# Autodesk Inventor assembly: Catapult Launcher
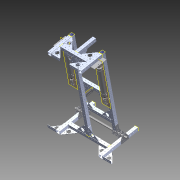
[picture p0: Inventor's stored thumbnail of the model, 180x180]
Saved by Autodesk Inventor 2014 (Build 180170000, 170)
## iProperties
Created: 2014-01-17
Part Number: Catapult Launcher
Document SubType Name: Assembly
Designer: Andrew Toennies
Mass: 1552.27 g
Surface Area: 5150.08 cm^2
Volume: 383.1 cm^3
Density: 4.05187 g/cm^3
Author: Andrew Toennies
## Documents named in this file (18)
- C:\Users\Andrew Toennies\Documents\GitHub\2014buildCAD\New Shooter\Catapult Launcher.iam
- C:\Users\Andrew Toennies\Documents\GitHub\2014buildCAD\New Shooter\Vex Pro 1x1 rectangular tubing 7 in length.ipt
- C:\Users\Andrew Toennies\Documents\GitHub\2014buildCAD\New Shooter\Vex Pro Side Bearing Gusset - OUT OF STOCK 1192014.ipt
- C:\Users\Andrew Toennies\Documents\GitHub\2014buildCAD\New Shooter\Vex Pro Corner Gusset - IN STOCK 1192014.ipt
- C:\Users\Andrew Toennies\Documents\GitHub\2014buildCAD\New Shooter\Bearing ID 0.500 Hex OD 1.125.ipt
- C:\Users\Andrew Toennies\Documents\GitHub\2014buildCAD\New Shooter\Shaft (Steel 0.500 Hex).ipt
- C:\Users\Andrew Toennies\Documents\GitHub\2014buildCAD\New Shooter\Vex Pro 1x1 rectangular tubing 27 in length.ipt
- C:\Users\Andrew Toennies\Documents\GitHub\2014buildCAD\New Shooter\Vex Pro 1x1 rectangular tubing 3 in length.ipt
- C:\Users\Andrew Toennies\Documents\GitHub\2014buildCAD\New Shooter\Vex Pro 1x1 rectangular tubing 11 in length.ipt
- C:\Users\Andrew Toennies\Documents\GitHub\2014buildCAD\New Shooter\1.5 in bore 6 in stroke cylinder - BIMBA\176-DP(D-229)(F,D-231-1).iam
- C:\Users\Andrew Toennies\Documents\GitHub\2014buildCAD\New Shooter\Aluminum Plate (0.125).ipt
- C:\Users\Andrew Toennies\Documents\GitHub\2014buildCAD\New Shooter\1.5 in bore 6 in stroke cylinder - BIMBA\D-14826.ipt
- C:\Users\Andrew Toennies\Documents\GitHub\2014buildCAD\New Shooter\1.5 in bore 6 in stroke cylinder - BIMBA\D-9969.ipt
- C:\Users\Andrew Toennies\Documents\GitHub\2014buildCAD\New Shooter\Vex Pro End Bearing Mount - IN STOCK 1192014.ipt
- C:\Users\Andrew Toennies\Documents\GitHub\2014buildCAD\New Shooter\Vex Pro 1x1 rectangular tubing 13 in length.ipt
- C:\Users\Andrew Toennies\Documents\GitHub\2014buildCAD\New Shooter\Vex Pro 1x1 rectangular tubing 25 in length.ipt
- C:\Users\Andrew Toennies\Documents\GitHub\2014buildCAD\New Shooter\0.5625 in bore 2 in stroke compact cylinder - BIMBA\FO-022.iam
- C:\Users\Andrew Toennies\Documents\GitHub\2014buildCAD\New Shooter\Vex Pro 1x1 rectangular tubing 8 in length.ipt
## Components (53 placed, 17 different names)
1. Shaft (Steel 0.500 Hex):1 — Mate:34, Mate:35, Flush:25, Mate:227, Mate:228
2. Vex Pro 1x1 rectangular tubing 11 in length:3 — Mate:272, Flush:48, Mate:274, Flush:49, Mate:277, Flush:50, Mate:290, Mate:291, Mate:293, Flush:57, Mate:298, Flush:60
3. Vex Pro Corner Gusset - IN STOCK 1192014:15 — Mate:273, Mate:274, Flush:49, Mate:275
4. Vex Pro Corner Gusset - IN STOCK 1192014:16 — Mate:276, Mate:277, Flush:50
5. Vex Pro 1x1 rectangular tubing 13 in length:1 — Mate:278, Flush:51, Mate:280, Flush:52, Mate:281, Mate:284, Flush:55, Mate:294, Mate:296
6. Vex Pro 1x1 rectangular tubing 25 in length:1 — Mate:284, Flush:55, Mate:285, Mate:287, Mate:288, Mate:289, Flush:56, Mate:292, Mate:295, Flush:58, Mate:297, Flush:59, Flush:61, Mate:300
7. FO-022:1 [sub-assembly] — Mate:285, Mate:287, Mate:288
8. Vex Pro Corner Gusset - IN STOCK 1192014:17 — Mate:289, Mate:290, Flush:56, Mate:291
9. Vex Pro Corner Gusset - IN STOCK 1192014:18 — Mate:292, Mate:293, Flush:57
10. Vex Pro Corner Gusset - IN STOCK 1192014:19 — Mate:294, Mate:295, Flush:58
11. Vex Pro Corner Gusset - IN STOCK 1192014:20 — Mate:296, Mate:297, Flush:59
12. Vex Pro 1x1 rectangular tubing 8 in length:1 — Mate:298, Flush:60, Flush:61, Mate:299, Flush:62
13. Vex Pro Corner Gusset - IN STOCK 1192014:21 — Mate:299, Mate:300, Flush:62
14. Vex Pro 1x1 rectangular tubing 7 in length:1 — Flush:1, Flush:2, Mate:8, Mate:11, Mate:23, Mate:24, Mate:25, Mate:195, Flush:32, Flush:33, Flush:34, Flush:35, Mate:278, Flush:51, Mate:279
15. Vex Pro 1x1 rectangular tubing 7 in length:2 — Flush:1, Flush:2, Mate:3, Mate:5, Mate:14, Mate:15, Mate:16, Mate:123, Mate:188, Mate:195, Flush:25, Flush:28, Flush:29, Flush:30, Flush:31, Mate:282, Flush:54, Mate:283
16. Vex Pro Side Bearing Gusset - OUT OF STOCK 1192014:1 — Mate:3, Mate:26, Mate:27, Flush:28, Flush:29
17. Vex Pro Side Bearing Gusset - OUT OF STOCK 1192014:2 — Mate:5, Mate:28, Mate:29, Flush:30, Flush:31
18. Vex Pro Side Bearing Gusset - OUT OF STOCK 1192014:3 — Mate:11, Mate:32, Mate:33, Flush:32, Flush:33
19. Vex Pro Side Bearing Gusset - OUT OF STOCK 1192014:4 — Mate:8, Mate:30, Mate:31, Flush:34, Flush:35
20. Vex Pro Corner Gusset - IN STOCK 1192014:1 — Mate:281, Mate:282, Flush:54, Mate:283
21. Vex Pro Corner Gusset - IN STOCK 1192014:2 — Mate:14, Mate:15, Mate:16, Flush:53
22. Vex Pro Corner Gusset - IN STOCK 1192014:3 — Mate:279, Mate:280, Flush:52
23. Vex Pro Corner Gusset - IN STOCK 1192014:4 — Mate:23, Mate:24, Mate:25
24. Bearing ID 0.500 Hex OD 1.125:1 — Mate:28, Mate:29, Flush:3, Flush:5
25. Bearing ID 0.500 Hex OD 1.125:2 — Mate:26, Mate:27, Flush:3, Mate:34, Mate:35
26. Bearing ID 0.500 Hex OD 1.125:3 — Mate:30, Mate:31, Flush:4
27. Bearing ID 0.500 Hex OD 1.125:4 — Mate:32, Mate:33, Flush:4, Flush:5, Mate:69
28. Vex Pro Corner Gusset - IN STOCK 1192014:14 — Mate:250, Mate:251, Flush:45, Mate:271
29. Vex Pro Corner Gusset - IN STOCK 1192014:13 — Mate:252, Mate:253, Flush:46
30. Vex Pro Corner Gusset - IN STOCK 1192014:12 — Mate:248, Mate:249, Flush:44
31. Vex Pro Corner Gusset - IN STOCK 1192014:11 — Mate:243, Flush:43, Mate:244
32. Vex Pro 1x1 rectangular tubing 11 in length:1 — Mate:191, Flush:42, Mate:250, Mate:253, Flush:46, Mate:267
33. Vex Pro 1x1 rectangular tubing 11 in length:2 — Flush:41, Mate:242, Mate:243, Flush:43, Mate:246, Mate:248, Flush:44
34. D-9969:1 — Mate:164, Mate:165, Mate:166, Mate:198, Flush:36, Mate:270
35. D-14826:1 — Mate:164, Mate:169, Mate:170, Flush:37, Mate:247, Mate:265, Mate:266
36. Vex Pro End Bearing Mount - IN STOCK 1192014:4 — Mate:229, Mate:230, Mate:231, Mate:232, Mate:246
37. Vex Pro End Bearing Mount - IN STOCK 1192014:3 — Mate:217, Mate:218, Mate:219, Mate:220, Mate:221
38. Vex Pro End Bearing Mount - IN STOCK 1192014:2 — Mate:233, Mate:234, Mate:235, Mate:236, Mate:245
39. Vex Pro End Bearing Mount - IN STOCK 1192014:1 — Mate:222, Mate:223, Mate:224, Mate:225, Mate:226
40. Vex Pro 1x1 rectangular tubing 27 in length:3 — Mate:198, Mate:229, Mate:230, Mate:231, Mate:233, Mate:234, Mate:235, Flush:27, Flush:36, Flush:41, Mate:242, Mate:244, Mate:251, Flush:45, Mate:267, Mate:270, Mate:271
41. Vex Pro 1x1 rectangular tubing 27 in length:2 — Mate:188, Mate:191, Mate:212, Mate:219, Mate:220, Mate:221, Mate:224, Mate:225, Mate:226, Flush:26, Flush:37, Flush:42, Mate:247, Mate:249, Mate:252
42. Bearing ID 0.500 Hex OD 1.125:5 — Mate:80, Mate:222, Mate:223, Mate:228
43. Bearing ID 0.500 Hex OD 1.125:6 — Mate:80, Mate:217, Mate:218, Mate:227
44. Bearing ID 0.500 Hex OD 1.125:7 — Mate:68, Mate:69, Mate:236, Mate:245
45. Bearing ID 0.500 Hex OD 1.125:8 — Mate:68, Mate:232
46. 176-DP(D-229)(F,D-231-1):1 [sub-assembly] — Mate:153, Mate:154, Mate:155, Mate:165, Mate:166, Mate:171
47. 176-DP(D-229)(F,D-231-1):2 [sub-assembly] — Mate:156, Mate:167, Mate:168, Mate:169, Mate:170, Mate:171, Mate:265, Mate:266
48. Aluminum Plate (0.125):1 — Mate:153, Mate:154, Mate:155, Mate:159, Flush:24
49. Aluminum Plate (0.125):2 — Mate:156, Mate:160, Mate:167, Mate:168, Flush:24, Flush:47
50. Vex Pro 1x1 rectangular tubing 3 in length:2 — Mate:121, Flush:14, Mate:122, Flush:19, Mate:159, Flush:27, Mate:276
51. Vex Pro 1x1 rectangular tubing 3 in length:1 — Flush:13, Mate:118, Mate:119, Mate:120, Mate:123, Flush:19, Mate:160, Mate:212, Flush:26, Flush:47, Mate:272, Flush:48, Mate:273, Mate:275
52. Vex Pro Corner Gusset - IN STOCK 1192014:8 — Flush:13, Mate:118, Mate:119, Mate:120, Flush:17, Flush:53
53. Vex Pro Corner Gusset - IN STOCK 1192014:6 — Mate:121, Flush:14, Mate:122, Flush:17
## Relationships (158: Mate 113, Flush 45)
- Flush:1: Vex Pro 1x1 rectangular tubing 7 in length:1 ↔ Vex Pro 1x1 rectangular tubing 7 in length:2
- Flush:2: Vex Pro 1x1 rectangular tubing 7 in length:1 ↔ Vex Pro 1x1 rectangular tubing 7 in length:2
- Mate:3: Vex Pro 1x1 rectangular tubing 7 in length:2 ↔ Vex Pro Side Bearing Gusset - OUT OF STOCK 1192014:1
- Mate:5: Vex Pro 1x1 rectangular tubing 7 in length:2 ↔ Vex Pro Side Bearing Gusset - OUT OF STOCK 1192014:2
- Mate:8: Vex Pro 1x1 rectangular tubing 7 in length:1 ↔ Vex Pro Side Bearing Gusset - OUT OF STOCK 1192014:4
- Mate:11: Vex Pro 1x1 rectangular tubing 7 in length:1 ↔ Vex Pro Side Bearing Gusset - OUT OF STOCK 1192014:3
- Mate:14: Vex Pro 1x1 rectangular tubing 7 in length:2 ↔ Vex Pro Corner Gusset - IN STOCK 1192014:2
- Mate:15: Vex Pro 1x1 rectangular tubing 7 in length:2 ↔ Vex Pro Corner Gusset - IN STOCK 1192014:2
- Mate:16: Vex Pro 1x1 rectangular tubing 7 in length:2 ↔ Vex Pro Corner Gusset - IN STOCK 1192014:2
- Mate:23: Vex Pro 1x1 rectangular tubing 7 in length:1 ↔ Vex Pro Corner Gusset - IN STOCK 1192014:4
- Mate:24: Vex Pro 1x1 rectangular tubing 7 in length:1 ↔ Vex Pro Corner Gusset - IN STOCK 1192014:4
- Mate:25: Vex Pro 1x1 rectangular tubing 7 in length:1 ↔ Vex Pro Corner Gusset - IN STOCK 1192014:4
- Mate:26: Vex Pro Side Bearing Gusset - OUT OF STOCK 1192014:1 ↔ Bearing ID 0.500 Hex OD 1.125:2
- Mate:27: Vex Pro Side Bearing Gusset - OUT OF STOCK 1192014:1 ↔ Bearing ID 0.500 Hex OD 1.125:2
- Mate:28: Vex Pro Side Bearing Gusset - OUT OF STOCK 1192014:2 ↔ Bearing ID 0.500 Hex OD 1.125:1
- Mate:29: Vex Pro Side Bearing Gusset - OUT OF STOCK 1192014:2 ↔ Bearing ID 0.500 Hex OD 1.125:1
- Flush:3: Bearing ID 0.500 Hex OD 1.125:1 ↔ Bearing ID 0.500 Hex OD 1.125:2
- Mate:30: Vex Pro Side Bearing Gusset - OUT OF STOCK 1192014:4 ↔ Bearing ID 0.500 Hex OD 1.125:3
- Mate:31: Vex Pro Side Bearing Gusset - OUT OF STOCK 1192014:4 ↔ Bearing ID 0.500 Hex OD 1.125:3
- Mate:32: Vex Pro Side Bearing Gusset - OUT OF STOCK 1192014:3 ↔ Bearing ID 0.500 Hex OD 1.125:4
- Mate:33: Vex Pro Side Bearing Gusset - OUT OF STOCK 1192014:3 ↔ Bearing ID 0.500 Hex OD 1.125:4
- Flush:4: Bearing ID 0.500 Hex OD 1.125:3 ↔ Bearing ID 0.500 Hex OD 1.125:4
- Flush:5: Bearing ID 0.500 Hex OD 1.125:1 ↔ Bearing ID 0.500 Hex OD 1.125:4
- Mate:34: Shaft (Steel 0.500 Hex):1 ↔ Bearing ID 0.500 Hex OD 1.125:2
- Mate:35: Shaft (Steel 0.500 Hex):1 ↔ Bearing ID 0.500 Hex OD 1.125:2
- Mate:68: Bearing ID 0.500 Hex OD 1.125:7 ↔ Bearing ID 0.500 Hex OD 1.125:8
- Mate:69: Bearing ID 0.500 Hex OD 1.125:4 ↔ Bearing ID 0.500 Hex OD 1.125:7
- Mate:80: Bearing ID 0.500 Hex OD 1.125:5 ↔ Bearing ID 0.500 Hex OD 1.125:6
- Flush:13: Vex Pro 1x1 rectangular tubing 3 in length:1 ↔ Vex Pro Corner Gusset - IN STOCK 1192014:8
- Mate:118: Vex Pro 1x1 rectangular tubing 3 in length:1 ↔ Vex Pro Corner Gusset - IN STOCK 1192014:8
- Mate:119: Vex Pro 1x1 rectangular tubing 3 in length:1 ↔ Vex Pro Corner Gusset - IN STOCK 1192014:8
- Mate:120: Vex Pro 1x1 rectangular tubing 3 in length:1 ↔ Vex Pro Corner Gusset - IN STOCK 1192014:8
- Mate:121: Vex Pro 1x1 rectangular tubing 3 in length:2 ↔ Vex Pro Corner Gusset - IN STOCK 1192014:6
- Flush:14: Vex Pro 1x1 rectangular tubing 3 in length:2 ↔ Vex Pro Corner Gusset - IN STOCK 1192014:6
- Mate:122: Vex Pro 1x1 rectangular tubing 3 in length:2 ↔ Vex Pro Corner Gusset - IN STOCK 1192014:6
- Flush:17: Vex Pro Corner Gusset - IN STOCK 1192014:8 ↔ Vex Pro Corner Gusset - IN STOCK 1192014:6
- Mate:123 (-685.8 mm): Vex Pro 1x1 rectangular tubing 7 in length:2 ↔ Vex Pro 1x1 rectangular tubing 3 in length:1
- Flush:19: Vex Pro 1x1 rectangular tubing 3 in length:2 ↔ Vex Pro 1x1 rectangular tubing 3 in length:1
- Mate:153: 176-DP(D-229)(F,D-231-1):1 ↔ Aluminum Plate (0.125):1
- Mate:154: 176-DP(D-229)(F,D-231-1):1 ↔ Aluminum Plate (0.125):1
- Mate:155: 176-DP(D-229)(F,D-231-1):1 ↔ Aluminum Plate (0.125):1
- Mate:156: 176-DP(D-229)(F,D-231-1):2 ↔ Aluminum Plate (0.125):2
- Mate:159: Aluminum Plate (0.125):1 ↔ Vex Pro 1x1 rectangular tubing 3 in length:2
- Mate:160: Aluminum Plate (0.125):2 ↔ Vex Pro 1x1 rectangular tubing 3 in length:1
- Mate:164: D-9969:1 ↔ D-14826:1
- Mate:165: D-9969:1 ↔ 176-DP(D-229)(F,D-231-1):1
- Mate:166 (3.2131 mm): D-9969:1 ↔ 176-DP(D-229)(F,D-231-1):1
- Mate:167: 176-DP(D-229)(F,D-231-1):2 ↔ Aluminum Plate (0.125):2
- Mate:168: 176-DP(D-229)(F,D-231-1):2 ↔ Aluminum Plate (0.125):2
- Mate:169: D-14826:1 ↔ 176-DP(D-229)(F,D-231-1):2
- Mate:170 (3.2131 mm): D-14826:1 ↔ 176-DP(D-229)(F,D-231-1):2
- Mate:171: 176-DP(D-229)(F,D-231-1):1 ↔ 176-DP(D-229)(F,D-231-1):2
- Flush:24: Aluminum Plate (0.125):1 ↔ Aluminum Plate (0.125):2
- Mate:188 (25.4 mm): Vex Pro 1x1 rectangular tubing 7 in length:2 ↔ Vex Pro 1x1 rectangular tubing 27 in length:2
- Mate:191: Vex Pro 1x1 rectangular tubing 11 in length:1 ↔ Vex Pro 1x1 rectangular tubing 27 in length:2
- Mate:195 (330.2 mm): Vex Pro 1x1 rectangular tubing 7 in length:1 ↔ Vex Pro 1x1 rectangular tubing 7 in length:2
- Flush:25 (-25.4 mm): Shaft (Steel 0.500 Hex):1 ↔ Vex Pro 1x1 rectangular tubing 7 in length:2
- Mate:198: D-9969:1 ↔ Vex Pro 1x1 rectangular tubing 27 in length:3
- Mate:212: Vex Pro 1x1 rectangular tubing 27 in length:2 ↔ Vex Pro 1x1 rectangular tubing 3 in length:1
- Mate:217: Vex Pro End Bearing Mount - IN STOCK 1192014:3 ↔ Bearing ID 0.500 Hex OD 1.125:6
- Mate:218: Vex Pro End Bearing Mount - IN STOCK 1192014:3 ↔ Bearing ID 0.500 Hex OD 1.125:6
- Mate:219: Vex Pro End Bearing Mount - IN STOCK 1192014:3 ↔ Vex Pro 1x1 rectangular tubing 27 in length:2
- Mate:220: Vex Pro End Bearing Mount - IN STOCK 1192014:3 ↔ Vex Pro 1x1 rectangular tubing 27 in length:2
- Mate:221: Vex Pro End Bearing Mount - IN STOCK 1192014:3 ↔ Vex Pro 1x1 rectangular tubing 27 in length:2
- Mate:222: Vex Pro End Bearing Mount - IN STOCK 1192014:1 ↔ Bearing ID 0.500 Hex OD 1.125:5
- Mate:223: Vex Pro End Bearing Mount - IN STOCK 1192014:1 ↔ Bearing ID 0.500 Hex OD 1.125:5
- Mate:224: Vex Pro End Bearing Mount - IN STOCK 1192014:1 ↔ Vex Pro 1x1 rectangular tubing 27 in length:2
- Mate:225: Vex Pro End Bearing Mount - IN STOCK 1192014:1 ↔ Vex Pro 1x1 rectangular tubing 27 in length:2
- Mate:226: Vex Pro End Bearing Mount - IN STOCK 1192014:1 ↔ Vex Pro 1x1 rectangular tubing 27 in length:2
- Mate:227: Shaft (Steel 0.500 Hex):1 ↔ Bearing ID 0.500 Hex OD 1.125:6
- Mate:228: Shaft (Steel 0.500 Hex):1 ↔ Bearing ID 0.500 Hex OD 1.125:5
- Mate:229: Vex Pro End Bearing Mount - IN STOCK 1192014:4 ↔ Vex Pro 1x1 rectangular tubing 27 in length:3
- Mate:230: Vex Pro End Bearing Mount - IN STOCK 1192014:4 ↔ Vex Pro 1x1 rectangular tubing 27 in length:3
- Mate:231: Vex Pro End Bearing Mount - IN STOCK 1192014:4 ↔ Vex Pro 1x1 rectangular tubing 27 in length:3
- Mate:232: Vex Pro End Bearing Mount - IN STOCK 1192014:4 ↔ Bearing ID 0.500 Hex OD 1.125:8
- Mate:233: Vex Pro End Bearing Mount - IN STOCK 1192014:2 ↔ Vex Pro 1x1 rectangular tubing 27 in length:3
- Mate:234: Vex Pro End Bearing Mount - IN STOCK 1192014:2 ↔ Vex Pro 1x1 rectangular tubing 27 in length:3
- Mate:235: Vex Pro End Bearing Mount - IN STOCK 1192014:2 ↔ Vex Pro 1x1 rectangular tubing 27 in length:3
- Mate:236: Vex Pro End Bearing Mount - IN STOCK 1192014:2 ↔ Bearing ID 0.500 Hex OD 1.125:7
- Flush:26: Vex Pro 1x1 rectangular tubing 27 in length:2 ↔ Vex Pro 1x1 rectangular tubing 3 in length:1
- Flush:27: Vex Pro 1x1 rectangular tubing 27 in length:3 ↔ Vex Pro 1x1 rectangular tubing 3 in length:2
- Flush:28: Vex Pro 1x1 rectangular tubing 7 in length:2 ↔ Vex Pro Side Bearing Gusset - OUT OF STOCK 1192014:1
- Flush:29 (82.55 mm): Vex Pro 1x1 rectangular tubing 7 in length:2 ↔ Vex Pro Side Bearing Gusset - OUT OF STOCK 1192014:1
- Flush:30: Vex Pro 1x1 rectangular tubing 7 in length:2 ↔ Vex Pro Side Bearing Gusset - OUT OF STOCK 1192014:2
- Flush:31 (-82.55 mm): Vex Pro 1x1 rectangular tubing 7 in length:2 ↔ Vex Pro Side Bearing Gusset - OUT OF STOCK 1192014:2
- Flush:32: Vex Pro 1x1 rectangular tubing 7 in length:1 ↔ Vex Pro Side Bearing Gusset - OUT OF STOCK 1192014:3
- Flush:33 (82.55 mm): Vex Pro 1x1 rectangular tubing 7 in length:1 ↔ Vex Pro Side Bearing Gusset - OUT OF STOCK 1192014:3
- Flush:34: Vex Pro 1x1 rectangular tubing 7 in length:1 ↔ Vex Pro Side Bearing Gusset - OUT OF STOCK 1192014:4
- Flush:35 (-82.55 mm): Vex Pro 1x1 rectangular tubing 7 in length:1 ↔ Vex Pro Side Bearing Gusset - OUT OF STOCK 1192014:4
- Flush:36: D-9969:1 ↔ Vex Pro 1x1 rectangular tubing 27 in length:3
- Flush:37: D-14826:1 ↔ Vex Pro 1x1 rectangular tubing 27 in length:2
- Flush:41: Vex Pro 1x1 rectangular tubing 11 in length:2 ↔ Vex Pro 1x1 rectangular tubing 27 in length:3
- Mate:242: Vex Pro 1x1 rectangular tubing 11 in length:2 ↔ Vex Pro 1x1 rectangular tubing 27 in length:3
- Flush:42: Vex Pro 1x1 rectangular tubing 11 in length:1 ↔ Vex Pro 1x1 rectangular tubing 27 in length:2
- Mate:243: Vex Pro Corner Gusset - IN STOCK 1192014:11 ↔ Vex Pro 1x1 rectangular tubing 11 in length:2
- Flush:43: Vex Pro Corner Gusset - IN STOCK 1192014:11 ↔ Vex Pro 1x1 rectangular tubing 11 in length:2
- Mate:244: Vex Pro Corner Gusset - IN STOCK 1192014:11 ↔ Vex Pro 1x1 rectangular tubing 27 in length:3
- Mate:245: Vex Pro End Bearing Mount - IN STOCK 1192014:2 ↔ Bearing ID 0.500 Hex OD 1.125:7
- Mate:246 (6.35 mm): Vex Pro 1x1 rectangular tubing 11 in length:2 ↔ Vex Pro End Bearing Mount - IN STOCK 1192014:4
- Mate:247: D-14826:1 ↔ Vex Pro 1x1 rectangular tubing 27 in length:2
- Mate:248: Vex Pro Corner Gusset - IN STOCK 1192014:12 ↔ Vex Pro 1x1 rectangular tubing 11 in length:2
- Mate:249: Vex Pro Corner Gusset - IN STOCK 1192014:12 ↔ Vex Pro 1x1 rectangular tubing 27 in length:2
- Flush:44: Vex Pro Corner Gusset - IN STOCK 1192014:12 ↔ Vex Pro 1x1 rectangular tubing 11 in length:2
- Mate:250: Vex Pro Corner Gusset - IN STOCK 1192014:14 ↔ Vex Pro 1x1 rectangular tubing 11 in length:1
- Mate:251: Vex Pro Corner Gusset - IN STOCK 1192014:14 ↔ Vex Pro 1x1 rectangular tubing 27 in length:3
- Flush:45: Vex Pro Corner Gusset - IN STOCK 1192014:14 ↔ Vex Pro 1x1 rectangular tubing 27 in length:3
- Mate:252: Vex Pro Corner Gusset - IN STOCK 1192014:13 ↔ Vex Pro 1x1 rectangular tubing 27 in length:2
- Mate:253: Vex Pro Corner Gusset - IN STOCK 1192014:13 ↔ Vex Pro 1x1 rectangular tubing 11 in length:1
- Flush:46: Vex Pro Corner Gusset - IN STOCK 1192014:13 ↔ Vex Pro 1x1 rectangular tubing 11 in length:1
- Mate:265 (3.2131 mm): D-14826:1 ↔ 176-DP(D-229)(F,D-231-1):2
- Mate:266 (3.2131 mm): D-14826:1 ↔ 176-DP(D-229)(F,D-231-1):2
- Mate:267: Vex Pro 1x1 rectangular tubing 11 in length:1 ↔ Vex Pro 1x1 rectangular tubing 27 in length:3
- Flush:47: Aluminum Plate (0.125):2 ↔ Vex Pro 1x1 rectangular tubing 3 in length:1
- Mate:270: D-9969:1 ↔ Vex Pro 1x1 rectangular tubing 27 in length:3
- Mate:271: Vex Pro Corner Gusset - IN STOCK 1192014:14 ↔ Vex Pro 1x1 rectangular tubing 27 in length:3
- Mate:272: Vex Pro 1x1 rectangular tubing 11 in length:3 ↔ Vex Pro 1x1 rectangular tubing 3 in length:1
- Flush:48: Vex Pro 1x1 rectangular tubing 11 in length:3 ↔ Vex Pro 1x1 rectangular tubing 3 in length:1
- Mate:273: Vex Pro Corner Gusset - IN STOCK 1192014:15 ↔ Vex Pro 1x1 rectangular tubing 3 in length:1
- Mate:274: Vex Pro 1x1 rectangular tubing 11 in length:3 ↔ Vex Pro Corner Gusset - IN STOCK 1192014:15
- Flush:49: Vex Pro 1x1 rectangular tubing 11 in length:3 ↔ Vex Pro Corner Gusset - IN STOCK 1192014:15
- Mate:275: Vex Pro Corner Gusset - IN STOCK 1192014:15 ↔ Vex Pro 1x1 rectangular tubing 3 in length:1
- Mate:276: Vex Pro Corner Gusset - IN STOCK 1192014:16 ↔ Vex Pro 1x1 rectangular tubing 3 in length:2
- Mate:277: Vex Pro 1x1 rectangular tubing 11 in length:3 ↔ Vex Pro Corner Gusset - IN STOCK 1192014:16
- Flush:50: Vex Pro 1x1 rectangular tubing 11 in length:3 ↔ Vex Pro Corner Gusset - IN STOCK 1192014:16
- Mate:278: Vex Pro 1x1 rectangular tubing 13 in length:1 ↔ Vex Pro 1x1 rectangular tubing 7 in length:1
- Flush:51: Vex Pro 1x1 rectangular tubing 13 in length:1 ↔ Vex Pro 1x1 rectangular tubing 7 in length:1
- Mate:279: Vex Pro 1x1 rectangular tubing 7 in length:1 ↔ Vex Pro Corner Gusset - IN STOCK 1192014:3
- Mate:280: Vex Pro 1x1 rectangular tubing 13 in length:1 ↔ Vex Pro Corner Gusset - IN STOCK 1192014:3
- Flush:52: Vex Pro 1x1 rectangular tubing 13 in length:1 ↔ Vex Pro Corner Gusset - IN STOCK 1192014:3
- Flush:53: Vex Pro Corner Gusset - IN STOCK 1192014:2 ↔ Vex Pro Corner Gusset - IN STOCK 1192014:8
- Mate:281: Vex Pro 1x1 rectangular tubing 13 in length:1 ↔ Vex Pro Corner Gusset - IN STOCK 1192014:1
- Mate:282: Vex Pro 1x1 rectangular tubing 7 in length:2 ↔ Vex Pro Corner Gusset - IN STOCK 1192014:1
- Flush:54: Vex Pro 1x1 rectangular tubing 7 in length:2 ↔ Vex Pro Corner Gusset - IN STOCK 1192014:1
- Mate:283: Vex Pro 1x1 rectangular tubing 7 in length:2 ↔ Vex Pro Corner Gusset - IN STOCK 1192014:1
- Mate:284: Vex Pro 1x1 rectangular tubing 13 in length:1 ↔ Vex Pro 1x1 rectangular tubing 25 in length:1
- Flush:55: Vex Pro 1x1 rectangular tubing 13 in length:1 ↔ Vex Pro 1x1 rectangular tubing 25 in length:1
- Mate:285: Vex Pro 1x1 rectangular tubing 25 in length:1 ↔ FO-022:1
- Mate:287: Vex Pro 1x1 rectangular tubing 25 in length:1 ↔ FO-022:1
- Mate:288: Vex Pro 1x1 rectangular tubing 25 in length:1 ↔ FO-022:1
- Mate:289: Vex Pro 1x1 rectangular tubing 25 in length:1 ↔ Vex Pro Corner Gusset - IN STOCK 1192014:17
- Mate:290: Vex Pro 1x1 rectangular tubing 11 in length:3 ↔ Vex Pro Corner Gusset - IN STOCK 1192014:17
- Flush:56: Vex Pro 1x1 rectangular tubing 25 in length:1 ↔ Vex Pro Corner Gusset - IN STOCK 1192014:17
- Mate:291: Vex Pro 1x1 rectangular tubing 11 in length:3 ↔ Vex Pro Corner Gusset - IN STOCK 1192014:17
- Mate:292: Vex Pro 1x1 rectangular tubing 25 in length:1 ↔ Vex Pro Corner Gusset - IN STOCK 1192014:18
- Mate:293: Vex Pro 1x1 rectangular tubing 11 in length:3 ↔ Vex Pro Corner Gusset - IN STOCK 1192014:18
- Flush:57: Vex Pro 1x1 rectangular tubing 11 in length:3 ↔ Vex Pro Corner Gusset - IN STOCK 1192014:18
- Mate:294: Vex Pro 1x1 rectangular tubing 13 in length:1 ↔ Vex Pro Corner Gusset - IN STOCK 1192014:19
- Mate:295: Vex Pro 1x1 rectangular tubing 25 in length:1 ↔ Vex Pro Corner Gusset - IN STOCK 1192014:19
- Flush:58: Vex Pro 1x1 rectangular tubing 25 in length:1 ↔ Vex Pro Corner Gusset - IN STOCK 1192014:19
- Mate:296: Vex Pro 1x1 rectangular tubing 13 in length:1 ↔ Vex Pro Corner Gusset - IN STOCK 1192014:20
- Mate:297: Vex Pro 1x1 rectangular tubing 25 in length:1 ↔ Vex Pro Corner Gusset - IN STOCK 1192014:20
- Flush:59: Vex Pro 1x1 rectangular tubing 25 in length:1 ↔ Vex Pro Corner Gusset - IN STOCK 1192014:20
- Mate:298: Vex Pro 1x1 rectangular tubing 11 in length:3 ↔ Vex Pro 1x1 rectangular tubing 8 in length:1
- Flush:60: Vex Pro 1x1 rectangular tubing 11 in length:3 ↔ Vex Pro 1x1 rectangular tubing 8 in length:1
- Flush:61: Vex Pro 1x1 rectangular tubing 25 in length:1 ↔ Vex Pro 1x1 rectangular tubing 8 in length:1
- Mate:299: Vex Pro 1x1 rectangular tubing 8 in length:1 ↔ Vex Pro Corner Gusset - IN STOCK 1192014:21
- Mate:300: Vex Pro 1x1 rectangular tubing 25 in length:1 ↔ Vex Pro Corner Gusset - IN STOCK 1192014:21
- Flush:62: Vex Pro 1x1 rectangular tubing 8 in length:1 ↔ Vex Pro Corner Gusset - IN STOCK 1192014:21
